# Autodesk Inventor assembly: Assembly1
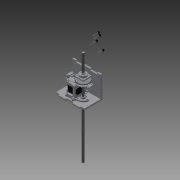
[picture p0: Inventor's stored thumbnail of the model, 180x180]
Saved by Autodesk Inventor 2015 (Build 190159000, 159)
## iProperties
Created: 2017-03-07
Part Number: Assembly1
Document SubType Name: Assembly
Designer: Ernest
Author: Ernest
## Documents named in this file (19)
- C:\Users\1esh9\Documents\Capstone-Project\doc\CAD\EndEffectorBase2\Assembly1.iam
- C:\Users\1esh9\Documents\Capstone-Project\doc\CAD\EndEffectorBase2\ThreadBar90.ipt
- C:\Users\1esh9\Documents\Capstone-Project\doc\CAD\Stepper Motor\NEMA-17\NEMA 17.iam
- C:\Users\1esh9\Documents\Capstone-Project\doc\CAD\Gears\Spur Gears1.iam
- C:\Users\1esh9\Documents\Capstone-Project\doc\CAD\Sensors\LineSensor.ipt
- C:\Users\1esh9\Documents\Capstone-Project\doc\CAD\Sensors\LinesensorHolderBottom.ipt
- C:\Users\1esh9\Documents\Capstone-Project\doc\CAD\Sensors\LinesensorHolderTop.ipt
- C:\Users\1esh9\Documents\Capstone-Project\doc\CAD\Sensors\LinesensorHolderWasher.ipt
- C:\Users\1esh9\Documents\Capstone-Project\doc\CAD\EndEffectorBase2\BigPositionDisk.ipt
- C:\Users\1esh9\Documents\Capstone-Project\doc\CAD\EndEffectorBase2\SmallPositionDisk.ipt
- C:\Users\1esh9\Documents\Capstone-Project\doc\CAD\LowLevel_Rev3\EE_base\EE_base_assembly.iam
- C:\Users\1esh9\Documents\Capstone-Project\doc\CAD\EndEffectorBase2\BallBearing.ipt
- C:\Users\1esh9\Documents\Capstone-Project\doc\CAD\EndEffectorBase2\BallBearingCenterer.ipt
- C:\Users\1esh9\Documents\Capstone-Project\doc\CAD\EndEffectorBase2\9mmRodNut.ipt
- C:\Users\1esh9\Documents\Capstone-Project\doc\CAD\EndEffectorBase2\BallBearingHolderTop.ipt
- C:\Users\1esh9\Documents\Capstone-Project\doc\CAD\EndEffectorBase2\BallBearingHolderBottom.ipt
- C:\Users\1esh9\Documents\Capstone-Project\doc\CAD\Sensors\TestMount.ipt
- C:\Users\1esh9\Documents\Capstone-Project\doc\CAD\EndEffectorBase2\MotorBracket.ipt
- C:\Users\1esh9\Documents\Capstone-Project\doc\CAD\Nuts and Bolts\SensorBolt-M3x11.ipt
## Components (31 placed, 18 different names)
1. ThreadBar90:1 — Mate:14, Mate:22, Mate:23, Mate:24, Mate:25, Mate:31, Mate:41, Mate:42, Mate:59, Mate:60
2. NEMA 17:1 [sub-assembly] — Mate:1, Mate:26, Angle:1, Mate:32, Mate:43, Mate:44, Mate:45, Mate:46, Angle:4, Mate:47, Mate:48, Mate:49, Mate:50, Mate:51, Mate:52, Mate:58
3. Spur Gears:1 [sub-assembly] — Mate:1, Mate:14, Mate:16, Mate:17, Mate:18, Mate:28, Mate:56
4. LineSensor:1
5. LineSensor:2
6. LineSensor:3
7. LineSensor:4
8. LinesensorHolderBottom:2 — Mate:5, Mate:6, Mate:7, Mate:43, Angle:4
9. LinesensorHolderTop:2 — Mate:2, Mate:3, Mate:4, Mate:5, Mate:7, Mate:38, Mate:39, Mate:40
10. LinesensorHolderWasher:1 — Mate:2, Mate:3, Mate:4, Mate:6
11. LinesensorHolderWasher:2 — Flush:5, Mate:59, Mate:60
12. BigPositionDisk:1 — Mate:31, Flush:5
13. SmallPositionDisk:1 — Mate:32, Mate:38, Mate:39, Mate:40
14. EE_base_assembly:1 [sub-assembly] — Mate:18, Flush:1, Angle:1, Angle:2, Mate:33, Mate:57, Angle:5
15. BallBearing:1 — Mate:16, Mate:20, Flush:3, Mate:27
16. BallBearing:2 — Mate:17, Flush:1, Mate:21, Flush:2, Mate:26
17. BallBearingCenterer:1 — Mate:20, Flush:3
18. BallBearingCenterer:2 — Mate:21, Flush:2
19. 9mmRodNut:1 — Mate:24
20. 9mmRodNut:2 — Mate:25
21. 9mmRodNut:3 — Mate:22
22. 9mmRodNut:4 — Mate:23
23. BallBearingHolderTop:1 — Mate:27, Mate:28, Angle:2, Mate:33
24. BallBearingHolderBottom:1 — Mate:56, Mate:57, Angle:5, Mate:58
25. 9mmRodNut:5 — Mate:41
26. 9mmRodNut:6 — Mate:42
27. TestMount:1 — Mate:44, Mate:45, Mate:46
28. MotorBracket:1 — Mate:48, Mate:50, Mate:52, Mate:55
29. MotorBracket:2 — Mate:47, Mate:49, Mate:51, Mate:53, Mate:54
30. SensorBolt-M3x11:1 — Flush:4, Mate:55
31. SensorBolt-M3x11:2 — Flush:4, Mate:53, Mate:54
## Relationships (55: Mate 46, Flush 5, Angle 4)
- Mate:1: NEMA 17:1 ↔ Spur Gears:1
- Mate:2: LinesensorHolderTop:2 ↔ LinesensorHolderWasher:1
- Mate:3: LinesensorHolderTop:2 ↔ LinesensorHolderWasher:1
- Mate:4: LinesensorHolderTop:2 ↔ LinesensorHolderWasher:1
- Mate:5: LinesensorHolderBottom:2 ↔ LinesensorHolderTop:2
- Mate:6: LinesensorHolderBottom:2 ↔ LinesensorHolderWasher:1
- Mate:7: LinesensorHolderBottom:2 ↔ LinesensorHolderTop:2
- Mate:14: ThreadBar90:1 ↔ Spur Gears:1
- Mate:16: Spur Gears:1 ↔ BallBearing:1
- Mate:17: Spur Gears:1 ↔ BallBearing:2
- Mate:18: Spur Gears:1 ↔ EE_base_assembly:1
- Flush:1: EE_base_assembly:1 ↔ BallBearing:2
- Mate:20: BallBearing:1 ↔ BallBearingCenterer:1
- Mate:21: BallBearing:2 ↔ BallBearingCenterer:2
- Flush:2 (0.4 mm): BallBearing:2 ↔ BallBearingCenterer:2
- Flush:3 (0.4 mm): BallBearing:1 ↔ BallBearingCenterer:1
- Mate:22: ThreadBar90:1 ↔ 9mmRodNut:3
- Mate:23: ThreadBar90:1 ↔ 9mmRodNut:4
- Mate:24: ThreadBar90:1 ↔ 9mmRodNut:1
- Mate:25: ThreadBar90:1 ↔ 9mmRodNut:2
- Mate:26 (5 mm): NEMA 17:1 ↔ BallBearing:2
- Angle:1 (0 deg): NEMA 17:1 ↔ EE_base_assembly:1
- Mate:27: BallBearing:1 ↔ BallBearingHolderTop:1
- Mate:28: Spur Gears:1 ↔ BallBearingHolderTop:1
- Angle:2 (0 deg): EE_base_assembly:1 ↔ BallBearingHolderTop:1
- Mate:31: ThreadBar90:1 ↔ BigPositionDisk:1
- Mate:32: NEMA 17:1 ↔ SmallPositionDisk:1
- Mate:33: EE_base_assembly:1 ↔ BallBearingHolderTop:1
- Mate:38 (0.2 mm): LinesensorHolderTop:2 ↔ SmallPositionDisk:1
- Mate:39 (26.387 mm): LinesensorHolderTop:2 ↔ SmallPositionDisk:1
- Mate:40 (26.387 mm): LinesensorHolderTop:2 ↔ SmallPositionDisk:1
- Mate:41: ThreadBar90:1 ↔ 9mmRodNut:5
- Mate:42: ThreadBar90:1 ↔ 9mmRodNut:6
- Mate:43 (3 mm): NEMA 17:1 ↔ LinesensorHolderBottom:2
- Mate:44: NEMA 17:1 ↔ TestMount:1
- Mate:45: NEMA 17:1 ↔ TestMount:1
- Mate:46: NEMA 17:1 ↔ TestMount:1
- Angle:4 (0 deg): NEMA 17:1 ↔ LinesensorHolderBottom:2
- Mate:47: NEMA 17:1 ↔ MotorBracket:2
- Mate:48: NEMA 17:1 ↔ MotorBracket:1
- Mate:49: NEMA 17:1 ↔ MotorBracket:2
- Mate:50: NEMA 17:1 ↔ MotorBracket:1
- Mate:51: NEMA 17:1 ↔ MotorBracket:2
- Mate:52: NEMA 17:1 ↔ MotorBracket:1
- Flush:4: SensorBolt-M3x11:1 ↔ SensorBolt-M3x11:2
- Mate:53: MotorBracket:2 ↔ SensorBolt-M3x11:2
- Mate:54: MotorBracket:2 ↔ SensorBolt-M3x11:2
- Mate:55: MotorBracket:1 ↔ SensorBolt-M3x11:1
- Mate:56: Spur Gears:1 ↔ BallBearingHolderBottom:1
- Mate:57: EE_base_assembly:1 ↔ BallBearingHolderBottom:1
- Angle:5 (0 deg): EE_base_assembly:1 ↔ BallBearingHolderBottom:1
- Mate:58: NEMA 17:1 ↔ BallBearingHolderBottom:1
- Flush:5 (-0.2 mm): LinesensorHolderWasher:2 ↔ BigPositionDisk:1
- Mate:59 (26.387 mm): ThreadBar90:1 ↔ LinesensorHolderWasher:2
- Mate:60 (26.387 mm): ThreadBar90:1 ↔ LinesensorHolderWasher:2
